# Autodesk Inventor assembly: 000-hand-grab-v4
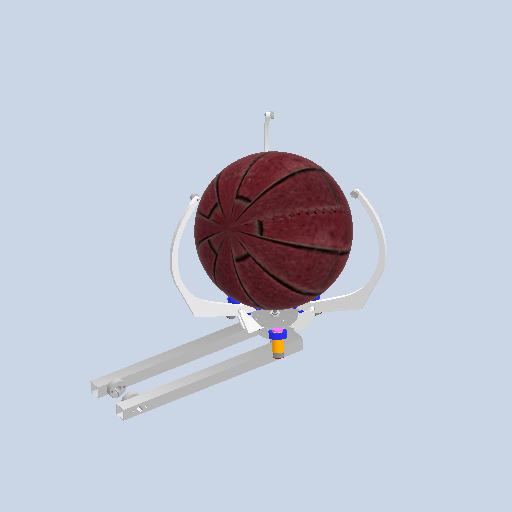
[picture p0: Inventor's stored thumbnail of the model, 512x512]
Saved by Autodesk Inventor 2025.2 (Build 292293000, 293)
## iProperties
Created: 2024-10-07
Part Number: 000-hand-grab-v4
Document SubType Name: Assembly
Designer: haruy
Author: haruy
## Documents named in this file (17)
- C:\Users\haruy\Documents\ロボコン\NHK2025\cad\nagahisa\hand\grab\000-hand-grab-v4.iam
- C:\Users\haruy\Documents\ロボコン\NHK2025\cad\nagahisa\hand\grab\hand-grab-v1-MDF-air-Base.ipt
- C:\Users\haruy\Documents\ロボコン\NHK2025\cad\nagahisa\hand\grab\hand-grab-v1-POM-link-F-1.ipt
- C:\Users\haruy\Documents\ロボコン\NHK2025\cad\nagahisa\hand\grab\hand-grab-v1-3DP-link-F-2.ipt
- C:\Users\haruy\Documents\ロボコン\NHK2025\cad\nagahisa\hand\grab\bearing-10-3.ipt
- C:\Users\haruy\Documents\ロボコン\NHK2025\cad\nagahisa\hand\grab\C-SEFL683ZZ.ipt
- C:\Users\haruy\Documents\ロボコン\NHK2025\cad\nagahisa\hand\grab\E-NTBGT13-8.iam
- C:\Users\haruy\Documents\ロボコン\NHK2025\cad\basket-ball.ipt
- C:\Users\haruy\Documents\ロボコン\NHK2025\cad\000_parts\エアシリンダー\airclinder\CDJ2B16-15Z-B(0_1_0).iam
- C:\Users\haruy\Documents\ロボコン\NHK2025\cad\nagahisa\hand\grab\hand-grab-v1-ASP-arm-support.ipt
- C:\Users\haruy\Documents\ロボコン\NHK2025\cad\nagahisa\hand\grab\hand-grab-v1-MDF-arm.ipt
- C:\Users\haruy\Documents\ロボコン\NHK2025\cad\nagahisa\hand\grab\hand-grab-v3-3DP-light_F.ipt
- C:\Users\haruy\Documents\ロボコン\NHK2025\cad\000_parts\センサー\E18_D80NK.ipt
- C:\Users\haruy\Documents\ロボコン\NHK2025\cad\nagahisa\hand\grab\hand-grab-v3-3DP-spesa_1.ipt
- C:\Users\haruy\Documents\ロボコン\NHK2025\cad\nagahisa\hand\grab\hand-grab-v3-Plate-ASP_F.ipt
- C:\Users\haruy\Documents\ロボコン\NHK2025\cad\nagahisa\hand\grab\hand-grab-v4-ASP_1.ipt
- C:\Users\haruy\Documents\ロボコン\NHK2025\cad\nagahisa\dribl\SCSW12-10.iam
## Components (44 placed, 16 different names)
1. hand-grab-v1-MDF-air-Base:1 — 挿入:2, 挿入:3, 挿入:4, 挿入:5, 挿入:6, 挿入:7, 挿入:8, 挿入:9, 挿入:10, 挿入:11, 挿入:12, 挿入:13, 挿入:30, 挿入:48, 挿入:64, 挿入:68, 挿入:69, 挿入:74, 挿入:75, 挿入:76, 挿入:77, 挿入:81
2. hand-grab-v1-POM-link-F-1:1 — 挿入:2, 挿入:3
3. hand-grab-v1-POM-link-F-1:2 — 挿入:4, 挿入:5
4. hand-grab-v1-POM-link-F-1:3 — 挿入:6, 挿入:7
5. hand-grab-v1-POM-link-F-1:4 — 挿入:8, 挿入:9
6. hand-grab-v1-POM-link-F-1:5 — 挿入:10, 挿入:11
7. hand-grab-v1-POM-link-F-1:6 — 挿入:12, 挿入:13, 角度:1, 挿入:80
8. hand-grab-v1-3DP-link-F-2:1 — 挿入:16, 挿入:18, 挿入:20, 角度:1, 挿入:31
9. bearing-10-3:1 — 挿入:15
10. bearing-10-3:2 — 挿入:15, 挿入:16, 正接:7
11. bearing-10-3:3
12. bearing-10-3:4 — 挿入:18
13. bearing-10-3:5 — 挿入:20
14. bearing-10-3:6
15. basket-ball:1 — 正接:6
16. CDJ2B16-15Z-B(0_1_0):1 [sub-assembly] — 挿入:30, 挿入:31
17. hand-grab-v1-ASP-arm-support:1
18. hand-grab-v1-ASP-arm-support:2
19. hand-grab-v3-3DP-light_F:1 — 挿入:44, 挿入:68, 挿入:69
20. hand-grab-v3-3DP-light_F:2 — 挿入:46, 挿入:74, 挿入:75
21. hand-grab-v3-3DP-light_F:3 — 挿入:45, 挿入:76, 挿入:77
22. E18_D80NK:1 — 挿入:44
23. E18_D80NK:2 — 挿入:46
24. E18_D80NK:3 — 挿入:45
25. hand-grab-v3-3DP-spesa_1:1 — 挿入:48
26. hand-grab-v3-3DP-spesa_1:2 — 挿入:81, 挿入:83
27. hand-grab-v3-3DP-spesa_1:3 — 挿入:64, 挿入:82
28. hand-grab-v3-Plate-ASP_F:1 — 挿入:82, 挿入:83, 挿入:84, 挿入:85, 挿入:86, 挿入:87
29. hand-grab-v4-ASP_1:1 — 挿入:58, 挿入:84, 挿入:85
30. hand-grab-v4-ASP_1:2 — 挿入:59, 挿入:86, 挿入:87
31. SCSW12-10:1 [sub-assembly] — 挿入:58
32. SCSW12-10:2 [sub-assembly] — 挿入:59
33. hand-grab-v1-MDF-arm:1 — 挿入:36, 挿入:78, 挿入:79, 正接:7
34. C-SEFL683ZZ:1 — 挿入:79, 挿入:80
35. C-SEFL683ZZ:2 — 挿入:78
36. E-NTBGT13-8:1 [sub-assembly] — 正接:6, 挿入:36
37. hand-grab-v1-MDF-arm:2
38. C-SEFL683ZZ:3
39. C-SEFL683ZZ:4
40. E-NTBGT13-8:2 [sub-assembly]
41. hand-grab-v1-MDF-arm:3
42. C-SEFL683ZZ:5
43. C-SEFL683ZZ:6
44. E-NTBGT13-8:3 [sub-assembly]
## Component patterns: (3 elements, first: hand-grab-v1-MDF-arm:1 + C-SEFL683ZZ:1 + C-SEFL683ZZ:2 + E-NTBGT13-8:1)
## Relationships (47: Insert 44, Tangent 2, Angle 1)
- 挿入:2 [Insert]: hand-grab-v1-MDF-air-Base:1 ↔ hand-grab-v1-POM-link-F-1:1
- 挿入:3 [Insert]: hand-grab-v1-MDF-air-Base:1 ↔ hand-grab-v1-POM-link-F-1:1
- 挿入:4 [Insert]: hand-grab-v1-MDF-air-Base:1 ↔ hand-grab-v1-POM-link-F-1:2
- 挿入:5 [Insert]: hand-grab-v1-MDF-air-Base:1 ↔ hand-grab-v1-POM-link-F-1:2
- 挿入:6 [Insert]: hand-grab-v1-MDF-air-Base:1 ↔ hand-grab-v1-POM-link-F-1:3
- 挿入:7 [Insert]: hand-grab-v1-MDF-air-Base:1 ↔ hand-grab-v1-POM-link-F-1:3
- 挿入:8 [Insert]: hand-grab-v1-MDF-air-Base:1 ↔ hand-grab-v1-POM-link-F-1:4
- 挿入:9 [Insert]: hand-grab-v1-MDF-air-Base:1 ↔ hand-grab-v1-POM-link-F-1:4
- 挿入:10 [Insert]: hand-grab-v1-MDF-air-Base:1 ↔ hand-grab-v1-POM-link-F-1:5
- 挿入:11 [Insert]: hand-grab-v1-MDF-air-Base:1 ↔ hand-grab-v1-POM-link-F-1:5
- 挿入:12 [Insert]: hand-grab-v1-MDF-air-Base:1 ↔ hand-grab-v1-POM-link-F-1:6
- 挿入:13 [Insert]: hand-grab-v1-MDF-air-Base:1 ↔ hand-grab-v1-POM-link-F-1:6
- 挿入:15 [Insert]: bearing-10-3:1 ↔ bearing-10-3:2
- 挿入:16 [Insert] (0.25 mm): hand-grab-v1-3DP-link-F-2:1 ↔ bearing-10-3:2
- [Insert]: bearing-10-3:3 ↔ bearing-10-3:4
- 挿入:18 [Insert] (0.25 mm): hand-grab-v1-3DP-link-F-2:1 ↔ bearing-10-3:4
- [Insert]: bearing-10-3:5 ↔ bearing-10-3:6
- 挿入:20 [Insert] (0.25 mm): hand-grab-v1-3DP-link-F-2:1 ↔ bearing-10-3:5
- 角度:1 [Angle] (0 deg): hand-grab-v1-POM-link-F-1:6 ↔ hand-grab-v1-3DP-link-F-2:1
- 挿入:30 [Insert]: hand-grab-v1-MDF-air-Base:1 ↔ CDJ2B16-15Z-B(0_1_0):1
- 正接:6 [Tangent]: basket-ball:1 ↔ E-NTBGT13-8:1
- 挿入:31 [Insert] (4 mm): hand-grab-v1-3DP-link-F-2:1 ↔ CDJ2B16-15Z-B(0_1_0):1
- 挿入:36 [Insert]: hand-grab-v1-MDF-arm:1 ↔ E-NTBGT13-8:1
- 挿入:44 [Insert]: hand-grab-v3-3DP-light_F:1 ↔ E18_D80NK:1
- 挿入:45 [Insert]: hand-grab-v3-3DP-light_F:3 ↔ E18_D80NK:3
- 挿入:46 [Insert]: hand-grab-v3-3DP-light_F:2 ↔ E18_D80NK:2
- 挿入:48 [Insert]: hand-grab-v1-MDF-air-Base:1 ↔ hand-grab-v3-3DP-spesa_1:1
- 挿入:58 [Insert]: hand-grab-v4-ASP_1:1 ↔ SCSW12-10:1
- 挿入:59 [Insert]: hand-grab-v4-ASP_1:2 ↔ SCSW12-10:2
- 挿入:64 [Insert]: hand-grab-v1-MDF-air-Base:1 ↔ hand-grab-v3-3DP-spesa_1:3
- 挿入:68 [Insert]: hand-grab-v1-MDF-air-Base:1 ↔ hand-grab-v3-3DP-light_F:1
- 挿入:69 [Insert]: hand-grab-v1-MDF-air-Base:1 ↔ hand-grab-v3-3DP-light_F:1
- 挿入:74 [Insert]: hand-grab-v1-MDF-air-Base:1 ↔ hand-grab-v3-3DP-light_F:2
- 挿入:75 [Insert]: hand-grab-v1-MDF-air-Base:1 ↔ hand-grab-v3-3DP-light_F:2
- 挿入:76 [Insert]: hand-grab-v1-MDF-air-Base:1 ↔ hand-grab-v3-3DP-light_F:3
- 挿入:77 [Insert]: hand-grab-v1-MDF-air-Base:1 ↔ hand-grab-v3-3DP-light_F:3
- 挿入:78 [Insert]: hand-grab-v1-MDF-arm:1 ↔ C-SEFL683ZZ:2
- 挿入:79 [Insert]: hand-grab-v1-MDF-arm:1 ↔ C-SEFL683ZZ:1
- 挿入:80 [Insert] (0.2 mm): hand-grab-v1-POM-link-F-1:6 ↔ C-SEFL683ZZ:1
- 正接:7 [Tangent]: bearing-10-3:2 ↔ hand-grab-v1-MDF-arm:1
- 挿入:81 [Insert]: hand-grab-v1-MDF-air-Base:1 ↔ hand-grab-v3-3DP-spesa_1:2
- 挿入:82 [Insert]: hand-grab-v3-3DP-spesa_1:3 ↔ hand-grab-v3-Plate-ASP_F:1
- 挿入:83 [Insert]: hand-grab-v3-3DP-spesa_1:2 ↔ hand-grab-v3-Plate-ASP_F:1
- 挿入:84 [Insert]: hand-grab-v3-Plate-ASP_F:1 ↔ hand-grab-v4-ASP_1:1
- 挿入:85 [Insert]: hand-grab-v3-Plate-ASP_F:1 ↔ hand-grab-v4-ASP_1:1
- 挿入:86 [Insert]: hand-grab-v3-Plate-ASP_F:1 ↔ hand-grab-v4-ASP_1:2
- 挿入:87 [Insert]: hand-grab-v3-Plate-ASP_F:1 ↔ hand-grab-v4-ASP_1:2
## Named parameters: d16_d14 = 0 mm, d18_d14 = 0 mm
